# Autodesk Inventor assembly: Ensemble2
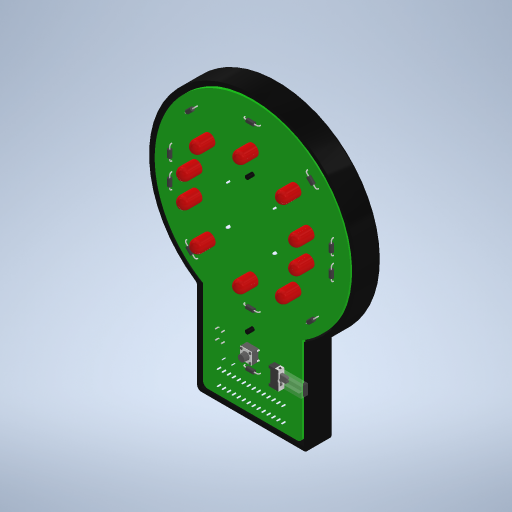
[picture p0: Inventor's stored thumbnail of the model, 512x512]
Saved by Autodesk Inventor 2024 (Build 280153000, 153)
## iProperties
Created: 2023-11-16
Part Number: Ensemble2
Document SubType Name: Assembly
Designer: digiacom
Author: digiacom
## Documents named in this file (5)
- D:\Projet\Perso\ATMegaSpin\Inventor\Ensemble2.iam
- D:\Projet\Perso\ATMegaSpin\Inventor\EnsemblePCB\EnsemblePCB.ipt
- D:\Projet\Perso\ATMegaSpin\Inventor\TopBox.ipt
- D:\Projet\Perso\ATMegaSpin\Inventor\BottomBox.ipt
- D:\Projet\Perso\ATMegaSpin\Inventor\SwitchOnOff.ipt
## Components (4 placed, 4 different names)
1. EnsemblePCB:1 — Affleurement:1, Affleurement:2, Placage:1, Placage:2
2. BottomBox:1 — Affleurement:1, Affleurement:2, Placage:1, Affleurement:3, Affleurement:4, Placage:3
3. TopBox:1 — Placage:2, Affleurement:3, Affleurement:4, Placage:3
4. SwitchOnOff:1
## Relationships (7: Flush 4, Mate 3)
- Affleurement:1 [Flush] (-1 mm): EnsemblePCB:1 ↔ BottomBox:1
- Affleurement:2 [Flush] (-1 mm): EnsemblePCB:1 ↔ BottomBox:1
- Placage:1 [Mate]: EnsemblePCB:1 ↔ BottomBox:1
- Placage:2 [Mate]: EnsemblePCB:1 ↔ TopBox:1
- Affleurement:3 [Flush]: BottomBox:1 ↔ TopBox:1
- Affleurement:4 [Flush]: BottomBox:1 ↔ TopBox:1
- Placage:3 [Mate]: BottomBox:1 ↔ TopBox:1
